# Autodesk Inventor assembly: Coluna_Suspensao_4-Cabos_Modelo2
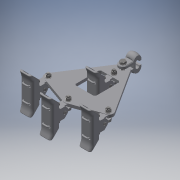
[picture p0: Inventor's stored thumbnail of the model, 180x180]
Saved by Autodesk Inventor 2018 (Build 220112000, 112)
## iProperties
Created: 2021-08-02
Part Number: Coluna_Suspensao_4-Cabos_Modelo2
Document SubType Name: Assembly
Designer: L08619
Author: L08619
## Documents named in this file (4)
- C:\Users\l08619\Documents\Projetos\TAESA\Modelo 3D - Tensionadores e Suspensão\Suporte de Suspenção\Coluna_Suspensao_4-Cabos_Modelo2.iam
- C:\Users\l08619\Documents\Projetos\TAESA\Modelo 3D - Tensionadores e Suspensão\Suporte de Suspenção\Corpo_Suporte_4_Cabos_Modelo2.ipt
- C:\Users\l08619\Documents\Projetos\TAESA\Modelo 3D - Tensionadores e Suspensão\Suporte de Suspenção\Clevis-Socket.iam
- C:\Users\l08619\Documents\Projetos\TAESA\Modelo 3D - Tensionadores e Suspensão\Suporte de Suspenção\Suspenssion_Clamp.iam
## Components (6 placed, 3 different names)
1. Corpo_Suporte_4_Cabos_Modelo2:1 — Mate:1, Mate:2, Cylindrical:1, Cylindrical:2, Cylindrical:3, Cylindrical:4, Cylindrical:5
2. Clevis-Socket:1 [sub-assembly] — Cylindrical:1
3. Suspenssion_Clamp:1 [sub-assembly] — Cylindrical:3
4. Suspenssion_Clamp:2 [sub-assembly] — Cylindrical:4
5. Suspenssion_Clamp:3 [sub-assembly] — Cylindrical:5
6. Suspenssion_Clamp:4 [sub-assembly] — Cylindrical:2
## Relationships (7: CylindricalJoint 5, Mate 2)
- Mate:1: Corpo_Suporte_4_Cabos_Modelo2:1
- Mate:2: Corpo_Suporte_4_Cabos_Modelo2:1
- Cylindrical:1: Corpo_Suporte_4_Cabos_Modelo2:1 ↔ Clevis-Socket:1
- Cylindrical:2: Corpo_Suporte_4_Cabos_Modelo2:1 ↔ Suspenssion_Clamp:4
- Cylindrical:3: Corpo_Suporte_4_Cabos_Modelo2:1 ↔ Suspenssion_Clamp:1
- Cylindrical:4: Corpo_Suporte_4_Cabos_Modelo2:1 ↔ Suspenssion_Clamp:2
- Cylindrical:5: Corpo_Suporte_4_Cabos_Modelo2:1 ↔ Suspenssion_Clamp:3
